# Autodesk Inventor assembly: üst şaft assembl
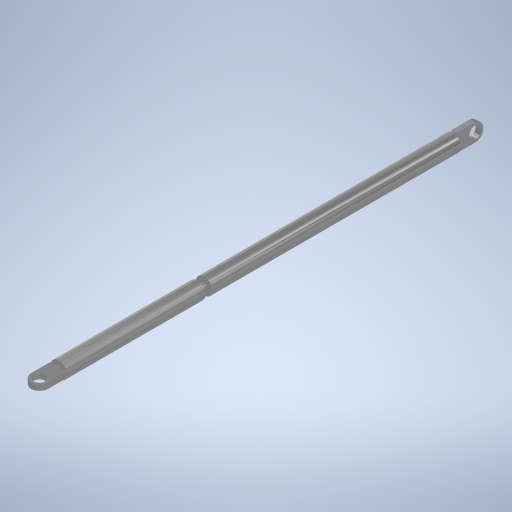
[picture p0: Inventor's stored thumbnail of the model, 512x512]
Saved by Autodesk Inventor 2023 (Build 270158000, 158)
## iProperties
Created: 2023-02-07
Part Number: üst şaft assembl
Document SubType Name: Assembly
Designer: omuru
Author: omuru
## Documents named in this file (3)
- C:\Users\omuru\Desktop\HUDSON süspansiyon + direksiyon sistemi\üst şaft assembl.iam
- C:\Users\omuru\Desktop\HUDSON süspansiyon + direksiyon sistemi\üst şaft part1.ipt
- C:\Users\omuru\Desktop\HUDSON süspansiyon + direksiyon sistemi\üst şaft part2.ipt
## Components (2 placed, 2 different names)
1. üst şaft part1:1 — Mate:1
2. üst şaft part2:1 — Mate:1
## Relationships (1: Mate 1)
- Mate:1: üst şaft part1:1 ↔ üst şaft part2:1
